# Autodesk Inventor assembly: Frame
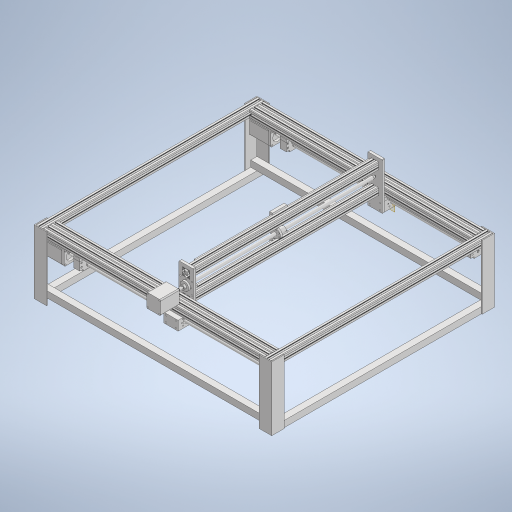
[picture p0: Inventor's stored thumbnail of the model, 512x512]
Saved by Autodesk Inventor 2023 (Build 270158000, 158)
## iProperties
Created: 2022-04-29
Part Number: Frame
Document SubType Name: Assembly
Designer: plebbb
Author: plebbb
## Documents named in this file (18)
- D:\Users\plebbb\Desktop\CNC_Project\Frame.iam
- D:\Users\plebbb\Desktop\CNC_Project\Frame_Gantry.iam
- D:\Users\plebbb\Desktop\CNC_Project\3030_Extrusion.ipt
- D:\Users\plebbb\Desktop\CNC_Project\Frame_Gantry_Reverse.iam
- D:\Users\plebbb\Desktop\CNC_Project\Frame_Gantry_Carrier.iam
- D:\Users\plebbb\Desktop\CNC_Project\Frame_Gantry_Carrier_Reverse.iam
- D:\Users\plebbb\Desktop\CNC_Project\Steel_Tube.ipt
- D:\Users\plebbb\Desktop\CNC_Project\Steel_Angle.ipt
- D:\Users\plebbb\Desktop\CNC_Project\Steel_Tube_longer.ipt
- D:\Users\plebbb\Desktop\CNC_Project\Y_Gantry_Connector.ipt
- D:\Users\plebbb\Desktop\CNC_Project\SFU1204-800.ipt
- D:\Users\plebbb\Desktop\CNC_Project\Y_Gantry_Connector_End.ipt
- D:\Users\plebbb\Desktop\CNC_Project\FK10.ipt
- D:\Users\plebbb\Desktop\CNC_Project\Nema23.ipt
- D:\Users\plebbb\Desktop\CNC_Project\3030_Extrusion_780.ipt
- D:\Users\plebbb\Desktop\CNC_Project\MGN15H-700.ipt
- D:\Users\plebbb\Desktop\CNC_Project\MGN15H-Carrier.ipt
- D:\Users\plebbb\Desktop\CNC_Project\SFU1204-Housing.ipt
## Components (26 placed, 17 different names)
1. Frame_Gantry:1 [sub-assembly] — Mate:1, Flush:1, Flush:2, Flush:3, Mate:7, Flush:15, Mate:19, Mate:47
2. 3030_Extrusion:2 — Mate:1, Flush:1, Flush:2, Mate:11, Flush:10, Flush:16, Mate:18, Mate:25, Flush:19
3. 3030_Extrusion:3 — Flush:3, Mate:7, Flush:9, Flush:5, Mate:9, Mate:20, Mate:21, Flush:17, Mate:22, Mate:23
4. Frame_Gantry_Reverse:1 [sub-assembly] — Flush:9, Flush:5, Mate:9, Mate:11, Flush:10, Flush:18, Mate:24
5. Frame_Gantry_Carrier:1 [sub-assembly] — Mate:42, Mate:43, Mate:44
6. Frame_Gantry_Carrier_Reverse:1 [sub-assembly] — Mate:38, Mate:39, Mate:40
7. Steel_Tube:1 — Mate:26, Mate:27, Flush:20, Mate:28
8. Steel_Angle:1 — Flush:16, Mate:18, Mate:19, Mate:27, Flush:20, Mate:28
9. Steel_Angle:2 — Mate:22, Mate:23, Flush:18, Mate:29, Mate:30, Mate:35, Mate:36, Mate:37
10. Steel_Angle:3 — Mate:20, Mate:21, Flush:17, Flush:21, Mate:31, Mate:33
11. Steel_Angle:4 — Mate:24, Mate:25, Flush:19, Mate:26
12. Steel_Tube:2 — Mate:29, Mate:30, Flush:21, Mate:32, Mate:34
13. Steel_Tube_longer:1 — Mate:31, Mate:32, Mate:33
14. Steel_Tube_longer:2 — Mate:34, Mate:35, Mate:36, Mate:37
15. Y_Gantry_Connector:1 — Mate:38, Mate:39, Mate:40, Mate:41, Mate:48, Angle:1, Flush:22, Flush:23, Mate:51, Mate:52, Mate:53, Mate:54, Mate:55, Mate:59
16. SFU1204-800:1 — Mate:41, Mate:45, Mate:46, Mate:49, Mate:50, Mate:65
17. Y_Gantry_Connector_End:1 — Mate:42, Mate:43, Mate:44, Mate:56, Mate:58
18. FK10:1 — Mate:45, Mate:46, Mate:48, Mate:59
19. Nema23:1 — Mate:49, Mate:50, Angle:1
20. 3030_Extrusion_780:1 — Flush:22, Mate:51, Mate:52, Mate:56, Mate:60, Flush:25
21. 3030_Extrusion_780:2 — Flush:23, Mate:53, Mate:54, Mate:55, Flush:24, Mate:57
22. MGN15H-700:1 — Flush:24, Mate:57, Mate:58, Flush:26, Mate:63, Mate:64, Flush:27
23. MGN15H-700:2 — Mate:60, Flush:25, Flush:26, Mate:61, Mate:62, Flush:28
24. MGN15H-Carrier:1 — Mate:63, Mate:64, Flush:27, Flush:29
25. MGN15H-Carrier:2 — Mate:61, Mate:62, Flush:28, Mate:66, Flush:29
26. SFU1204-Housing:1 — Mate:65, Mate:66
## Relationships (85: Mate 59, Flush 25, Angle 1)
- Mate:1: Frame_Gantry:1 ↔ 3030_Extrusion:2
- Flush:1: Frame_Gantry:1 ↔ 3030_Extrusion:2
- Flush:2: Frame_Gantry:1 ↔ 3030_Extrusion:2
- Flush:3: Frame_Gantry:1 ↔ 3030_Extrusion:3
- Mate:7: Frame_Gantry:1 ↔ 3030_Extrusion:3
- Flush:9: 3030_Extrusion:3 ↔ Frame_Gantry_Reverse:1
- Flush:5: 3030_Extrusion:3 ↔ Frame_Gantry_Reverse:1
- Mate:9: 3030_Extrusion:3 ↔ Frame_Gantry_Reverse:1
- Mate:11: 3030_Extrusion:2 ↔ Frame_Gantry_Reverse:1
- Flush:10: 3030_Extrusion:2 ↔ Frame_Gantry_Reverse:1
- [Flush] (-4 mm): Frame_Gantry:1 ↔ Frame_Gantry_Carrier:1
- [Mate]: Frame_Gantry:1 ↔ Frame_Gantry_Carrier:1
- [Flush]: Frame_Gantry:1 ↔ Frame_Gantry_Carrier:1
- [Mate]: Frame_Gantry:1 ↔ Frame_Gantry_Carrier:1
- [Mate]: Frame_Gantry:1 ↔ Frame_Gantry_Carrier:1
- [Flush] (-4 mm): Frame_Gantry_Reverse:1 ↔ Frame_Gantry_Carrier_Reverse:1
- [Mate]: Frame_Gantry_Reverse:1 ↔ Frame_Gantry_Carrier_Reverse:1
- [Flush]: Frame_Gantry_Reverse:1 ↔ Frame_Gantry_Carrier_Reverse:1
- [Mate]: Frame_Gantry_Reverse:1 ↔ Frame_Gantry_Carrier_Reverse:1
- [Mate]: Frame_Gantry_Reverse:1 ↔ Frame_Gantry_Carrier_Reverse:1
- Flush:15: Frame_Gantry:1
- Flush:16: 3030_Extrusion:2 ↔ Steel_Angle:1
- Mate:18: 3030_Extrusion:2 ↔ Steel_Angle:1
- Mate:19: Frame_Gantry:1 ↔ Steel_Angle:1
- Mate:20: 3030_Extrusion:3 ↔ Steel_Angle:3
- Mate:21: 3030_Extrusion:3 ↔ Steel_Angle:3
- Flush:17: 3030_Extrusion:3 ↔ Steel_Angle:3
- Mate:22: 3030_Extrusion:3 ↔ Steel_Angle:2
- Mate:23: 3030_Extrusion:3 ↔ Steel_Angle:2
- Flush:18: Frame_Gantry_Reverse:1 ↔ Steel_Angle:2
- Mate:24: Frame_Gantry_Reverse:1 ↔ Steel_Angle:4
- Mate:25: 3030_Extrusion:2 ↔ Steel_Angle:4
- Flush:19: 3030_Extrusion:2 ↔ Steel_Angle:4
- Mate:26: Steel_Tube:1 ↔ Steel_Angle:4
- Mate:27: Steel_Tube:1 ↔ Steel_Angle:1
- Flush:20: Steel_Tube:1 ↔ Steel_Angle:1
- Mate:28: Steel_Tube:1 ↔ Steel_Angle:1
- Mate:29: Steel_Angle:2 ↔ Steel_Tube:2
- Mate:30: Steel_Angle:2 ↔ Steel_Tube:2
- Flush:21: Steel_Angle:3 ↔ Steel_Tube:2
- Mate:31: Steel_Angle:3 ↔ Steel_Tube_longer:1
- Mate:32: Steel_Tube:2 ↔ Steel_Tube_longer:1
- Mate:33: Steel_Angle:3 ↔ Steel_Tube_longer:1
- Mate:34: Steel_Tube:2 ↔ Steel_Tube_longer:2
- Mate:35: Steel_Angle:2 ↔ Steel_Tube_longer:2
- Mate:36: Steel_Angle:2 ↔ Steel_Tube_longer:2
- Mate:37: Steel_Angle:2 ↔ Steel_Tube_longer:2
- Mate:38: Frame_Gantry_Carrier_Reverse:1 ↔ Y_Gantry_Connector:1
- Mate:39: Frame_Gantry_Carrier_Reverse:1 ↔ Y_Gantry_Connector:1
- Mate:40: Frame_Gantry_Carrier_Reverse:1 ↔ Y_Gantry_Connector:1
- Mate:41: Y_Gantry_Connector:1 ↔ SFU1204-800:1
- Mate:42: Frame_Gantry_Carrier:1 ↔ Y_Gantry_Connector_End:1
- Mate:43: Frame_Gantry_Carrier:1 ↔ Y_Gantry_Connector_End:1
- Mate:44: Frame_Gantry_Carrier:1 ↔ Y_Gantry_Connector_End:1
- Mate:45: SFU1204-800:1 ↔ FK10:1
- Mate:46: SFU1204-800:1 ↔ FK10:1
- Mate:47: Frame_Gantry:1
- Mate:48: Y_Gantry_Connector:1 ↔ FK10:1
- Mate:49: SFU1204-800:1 ↔ Nema23:1
- Mate:50: SFU1204-800:1 ↔ Nema23:1
- Angle:1 (0 deg): Y_Gantry_Connector:1 ↔ Nema23:1
- Flush:22: Y_Gantry_Connector:1 ↔ 3030_Extrusion_780:1
- Flush:23: Y_Gantry_Connector:1 ↔ 3030_Extrusion_780:2
- Mate:51: Y_Gantry_Connector:1 ↔ 3030_Extrusion_780:1
- Mate:52: Y_Gantry_Connector:1 ↔ 3030_Extrusion_780:1
- Mate:53: Y_Gantry_Connector:1 ↔ 3030_Extrusion_780:2
- Mate:54: Y_Gantry_Connector:1 ↔ 3030_Extrusion_780:2
- Mate:55: Y_Gantry_Connector:1 ↔ 3030_Extrusion_780:2
- Mate:56: Y_Gantry_Connector_End:1 ↔ 3030_Extrusion_780:1
- Flush:24 (7.5 mm): 3030_Extrusion_780:2 ↔ MGN15H-700:1
- Mate:57: 3030_Extrusion_780:2 ↔ MGN15H-700:1
- Mate:58: Y_Gantry_Connector_End:1 ↔ MGN15H-700:1
- Mate:59: Y_Gantry_Connector:1 ↔ FK10:1
- Mate:60: 3030_Extrusion_780:1 ↔ MGN15H-700:2
- Flush:25 (-7.5 mm): 3030_Extrusion_780:1 ↔ MGN15H-700:2
- Flush:26: MGN15H-700:1 ↔ MGN15H-700:2
- Mate:61: MGN15H-700:2 ↔ MGN15H-Carrier:2
- Mate:62: MGN15H-700:2 ↔ MGN15H-Carrier:2
- Mate:63: MGN15H-700:1 ↔ MGN15H-Carrier:1
- Mate:64: MGN15H-700:1 ↔ MGN15H-Carrier:1
- Flush:27: MGN15H-700:1 ↔ MGN15H-Carrier:1
- Flush:28: MGN15H-700:2 ↔ MGN15H-Carrier:2
- Mate:65: SFU1204-800:1 ↔ SFU1204-Housing:1
- Mate:66: MGN15H-Carrier:2 ↔ SFU1204-Housing:1
- Flush:29: MGN15H-Carrier:1 ↔ MGN15H-Carrier:2
## Named parameters: d13_d0 = 0 mm, d14_d2 = 0 mm, d15_d3 = 699 mm, d16_d4 = 0 mm, d3_d0 = -4 mm, d4_d1 = 0 mm, d5_d2 = 0 mm, d46_d3_d0 = -4 mm, d47_d4_d1 = 0 mm, d48_d5_d2 = 0 mm, d49_d3 = 651.2 mm, d50_d4 = 0 mm, d51_d13_d0 = 0 mm, d52_d14_d2 = 0 mm, d53_d15_d3 = 699 mm, d54_d16_d4 = 0 mm
